# Autodesk Inventor assembly: main
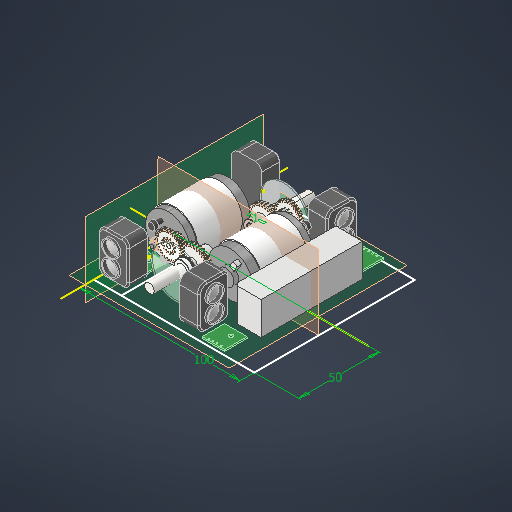
[picture p0: Inventor's stored thumbnail of the model, 512x512]
Saved by Autodesk Inventor 2026.2 (Build 302298000, 298)
## iProperties
Created: 2026-03-09
Part Number: main
Document SubType Name: Assembly
Designer: szymo
Author: szymo
## Documents named in this file (5)
- C:\Users\szymo\Downloads\evangelion-turbo\inventor-project\main.iam
- C:\Users\szymo\Downloads\evangelion-turbo\inventor-project\drive-train.iam
- C:\Users\szymo\Downloads\evangelion-turbo\inventor-project\LUNA.ipt
- C:\Users\szymo\Downloads\evangelion-turbo\inventor-project\3s450mah.ipt
- C:\Users\szymo\Downloads\evangelion-turbo\inventor-project\KTIR-Board.ipt
## Components (10 placed, 4 different names)
1. drive-train:1 [sub-assembly] — Flush:2, Flush:3, Flush:4, Mate:2, Mate:3, Tangent:1
2. 3s450mah:1 — Flush:8, Tangent:1, Flush:9
3. LUNA:2 — Mate:1, Mate:3, Angle:2, Flush:7
4. LUNA:1 — Flush:5, Mate:2, Angle:1, Flush:6
5. LUNA:3 — Flush:22, Flush:23, Mate:5, Mate:6
6. LUNA:4 — Flush:24, Flush:25, Flush:26, Mate:7
7. KTIR-Board:1 — Flush:10, Flush:11, Flush:13
8. KTIR-Board:2 — Mate:4, Flush:12, Flush:14
9. KTIR-Board:4 — Flush:17, Flush:27, Mate:6
10. KTIR-Board:5 — Flush:28, Flush:29, Mate:7
## Relationships (33: Flush 23, Mate 7, Angle 2, Tangent 1)
- Flush:1 (-101.75 mm)
- Flush:2 (0.65 mm): drive-train:1
- Flush:3 (-18.4 mm): drive-train:1
- Flush:4 (0.65 mm): drive-train:1
- Flush:5 (49.5 mm): LUNA:1
- Mate:1 (-49.5 mm): LUNA:2
- Mate:2 (18 mm): drive-train:1 ↔ LUNA:1
- Mate:3 (18 mm): drive-train:1 ↔ LUNA:2
- Angle:1 (0 deg): LUNA:1
- Angle:2 (180 deg): LUNA:2
- Flush:6 (2 mm): LUNA:1
- Flush:7 (2 mm): LUNA:2
- Flush:8 (2 mm): 3s450mah:1
- Tangent:1 (0.65 mm): drive-train:1 ↔ 3s450mah:1
- Flush:9 (-31 mm): 3s450mah:1
- Flush:10 (-49.5 mm): KTIR-Board:1
- Mate:4 (-49.5 mm): KTIR-Board:2
- Flush:11 (0.13 mm): KTIR-Board:1
- Flush:12 (0.13 mm): KTIR-Board:2
- Flush:13 (67 mm): KTIR-Board:1
- Flush:14 (-67 mm): KTIR-Board:2
- Flush:17: KTIR-Board:4
- Flush:22: LUNA:3
- Flush:23 (2 mm): LUNA:3
- Mate:5 (-49 mm): LUNA:3
- Flush:24 (2 mm): LUNA:4
- Flush:25: LUNA:4
- Flush:26 (-49 mm): LUNA:4
- Flush:27 (1 mm): KTIR-Board:4
- Flush:28 (1 mm): KTIR-Board:5
- Flush:29: KTIR-Board:5
- Mate:6 (1 mm): LUNA:3 ↔ KTIR-Board:4
- Mate:7 (1 mm): LUNA:4 ↔ KTIR-Board:5
